# Autodesk Inventor assembly: A04 - Acrylic Visor
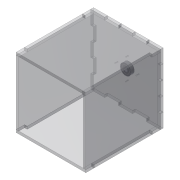
[picture p0: Inventor's stored thumbnail of the model, 180x180]
Saved by Autodesk Inventor 2016 (Build 200138000, 138)
## iProperties
Created: 2016-12-26
Part Number: A04 - Acrylic Visor
Document SubType Name: Conjunto soldado
Designer: Fernando
Weld Material: Aço macio soldado
Mass: 2242.71 g
Surface Area: 5024.5 cm^2
Volume: 1832.43 cm^3
Density: 1.2239 g/cm^3
SurfaceArea_m2: .5
Author: Fernando
## Documents named in this file (6)
- G:\00 - Files\00 - Personal\40 - Hobbies\90 - Projetos Particulares\40 - POV Display\01 - Mechanical Design\A04 - Acrylic Visor.iam
- G:\00 - Files\00 - Personal\40 - Hobbies\90 - Projetos Particulares\40 - POV Display\01 - Mechanical Design\M11 - Acrylic Top.ipt
- G:\00 - Files\00 - Personal\40 - Hobbies\90 - Projetos Particulares\40 - POV Display\01 - Mechanical Design\M12 - Acrylic Side 1.ipt
- G:\00 - Files\00 - Personal\40 - Hobbies\90 - Projetos Particulares\40 - POV Display\01 - Mechanical Design\M13 - Acrylic Side 2.ipt
- G:\00 - Files\00 - Personal\40 - Hobbies\90 - Projetos Particulares\40 - POV Display\01 - Mechanical Design\P03 - Bearing 62012.ipt
- G:\00 - Files\00 - Personal\40 - Hobbies\90 - Projetos Particulares\40 - POV Display\01 - Mechanical Design\M14 - Upper Bearing Support.ipt
## Components (8 placed, 5 different names)
1. M11 - Acrylic Top:1 — Flush:1, Flush:2, Flush:3, Flush:4, Flush:5, Flush:6, Flush:7, Flush:8, Flush:11, Insert:1, Mate:1, Mate:2
2. M12 - Acrylic Side 1:1 — Flush:1, Flush:2, Flush:3, Flush:9, Flush:12
3. M12 - Acrylic Side 1:2 — Flush:4, Flush:5, Flush:6, Flush:10
4. M13 - Acrylic Side 2:1 — Flush:7, Flush:8, Flush:9
5. M13 - Acrylic Side 2:2 — Flush:10, Flush:11, Flush:12
6. P03 - Bearing 62012:1 — Insert:1, Insert:2, Insert:3
7. M14 - Upper Bearing Support:1 — Insert:2, Mate:2
8. M14 - Upper Bearing Support:2 — Insert:3, Mate:1
## Relationships (17: Flush 12, Insert 3, Mate 2)
- Flush:1: M11 - Acrylic Top:1 ↔ M12 - Acrylic Side 1:1
- Flush:2: M11 - Acrylic Top:1 ↔ M12 - Acrylic Side 1:1
- Flush:3: M11 - Acrylic Top:1 ↔ M12 - Acrylic Side 1:1
- Flush:4: M11 - Acrylic Top:1 ↔ M12 - Acrylic Side 1:2
- Flush:5: M11 - Acrylic Top:1 ↔ M12 - Acrylic Side 1:2
- Flush:6: M11 - Acrylic Top:1 ↔ M12 - Acrylic Side 1:2
- Flush:7: M11 - Acrylic Top:1 ↔ M13 - Acrylic Side 2:1
- Flush:8: M11 - Acrylic Top:1 ↔ M13 - Acrylic Side 2:1
- Flush:9: M12 - Acrylic Side 1:1 ↔ M13 - Acrylic Side 2:1
- Flush:10: M12 - Acrylic Side 1:2 ↔ M13 - Acrylic Side 2:2
- Flush:11: M11 - Acrylic Top:1 ↔ M13 - Acrylic Side 2:2
- Flush:12: M12 - Acrylic Side 1:1 ↔ M13 - Acrylic Side 2:2
- Insert:1: M11 - Acrylic Top:1 ↔ P03 - Bearing 62012:1
- Insert:2: P03 - Bearing 62012:1 ↔ M14 - Upper Bearing Support:1
- Insert:3: P03 - Bearing 62012:1 ↔ M14 - Upper Bearing Support:2
- Mate:1: M11 - Acrylic Top:1 ↔ M14 - Upper Bearing Support:2
- Mate:2: M11 - Acrylic Top:1 ↔ M14 - Upper Bearing Support:1
